# Autodesk Inventor assembly: Skrzydło
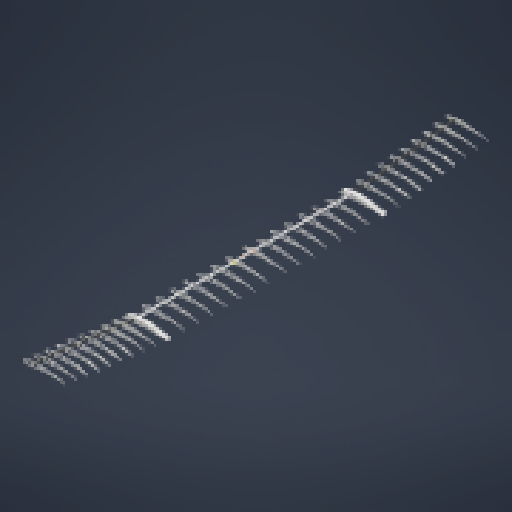
[picture p0: Inventor's stored thumbnail of the model, 512x512]
Saved by Autodesk Inventor 2023 (Build 270158000, 158)
## iProperties
Created: 2023-01-05
Part Number: Skrzydło
Document SubType Name: Assembly
Designer: szykr
Author: szykr
## Documents named in this file (6)
- D:\Folder Instalacyjny\GitHub Pliki\Solaris\new model\Skrzydło.iam
- D:\Folder Instalacyjny\GitHub Pliki\Solaris\new model\wingspar.ipt
- D:\Folder Instalacyjny\GitHub Pliki\Solaris\new model\Żerbo montaż.ipt
- D:\Folder Instalacyjny\GitHub Pliki\Solaris\new model\Żebro default.ipt
- D:\Folder Instalacyjny\GitHub Pliki\Solaris\new model\kuplung.ipt
- D:\Folder Instalacyjny\GitHub Pliki\Solaris\new model\skrzydlo_ster.iam
## Components (21 placed, 5 different names)
1. wingspar:1 — Insert:1, Insert:2
2. Żerbo montaż:1 — Insert:1, Insert:3, Insert:4
3. Żerbo montaż:2 — Insert:2, Insert:5, Insert:6
4. Żerbo montaż:3 — Insert:4, Insert:7
5. Żerbo montaż:4 — Insert:6, Insert:8
6. kuplung:1 — Insert:7, Insert:9
7. kuplung:2 — Insert:8, Insert:10
8. skrzydlo_ster:1 [sub-assembly] — Insert:9
9. skrzydlo_ster:2 [sub-assembly] — Insert:10
10. Żebro default:1 — Insert:3
11. Żebro default:2
12. Żebro default:3
13. Żebro default:4
14. Żebro default:5
15. Żebro default:6
16. Żebro default:7 — Insert:5
17. Żebro default:8
18. Żebro default:9
19. Żebro default:10
20. Żebro default:11
21. Żebro default:12
## Component patterns: (6 elements, first: Żebro default:1), (6 elements, first: Żebro default:7)
## Relationships (10: Insert 10)
- Insert:1 (-460 mm): wingspar:1 ↔ Żerbo montaż:1
- Insert:2 (-460 mm): wingspar:1 ↔ Żerbo montaż:2
- Insert:3 (-64.1429 mm): Żerbo montaż:1 ↔ Żebro default:1
- Insert:4 (449 mm): Żerbo montaż:1 ↔ Żerbo montaż:3
- Insert:5 (-64.1429 mm): Żerbo montaż:2 ↔ Żebro default:7
- Insert:6 (449 mm): Żerbo montaż:2 ↔ Żerbo montaż:4
- Insert:7: Żerbo montaż:3 ↔ kuplung:1
- Insert:8: Żerbo montaż:4 ↔ kuplung:2
- Insert:9: kuplung:1 ↔ skrzydlo_ster:1
- Insert:10: kuplung:2 ↔ skrzydlo_ster:2
## Named parameters: ilosc_cala_zeber = 8, ilosc_zeber_pattern = 6, dlugosc_zeber = 449 mm, spacing = 64.14286 mm
